# Autodesk Inventor assembly: Eje con costillas
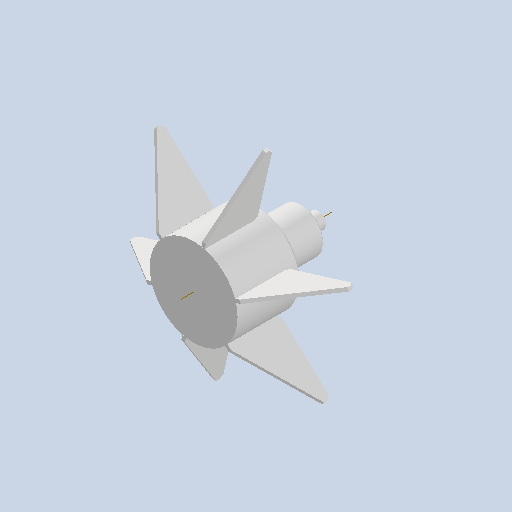
[picture p0: Inventor's stored thumbnail of the model, 512x512]
Saved by Autodesk Inventor 2024.3 (Build 283343000, 343)
## iProperties
Created: 2025-07-04
Part Number: Eje con costillas
Document SubType Name: Assembly
Designer: Daniel Rodriguez
Author: Daniel Rodriguez
## Documents named in this file (3)
- C:\Users\Daniel Rodriguez\Downloads\winch-drum-welding-assembly\Nuestro Winch\Eje con costillas.iam
- C:\Users\Daniel Rodriguez\Downloads\winch-drum-welding-assembly\Nuestro Winch\eje (bolt).ipt
- C:\Users\Daniel Rodriguez\Downloads\winch-drum-welding-assembly\Nuestro Winch\Costilla (rib).ipt
## Components (7 placed, 2 different names)
1. eje (bolt):1 — Nivelación:1, Tangente:1, Coincidencia:1
2. Costilla (rib):1 — Nivelación:1, Tangente:1
3. Costilla (rib):2
4. Costilla (rib):3
5. Costilla (rib):4
6. Costilla (rib):5
7. Costilla (rib):6
## Component patterns: (6 elements, first: Costilla (rib):1)
## Relationships (3: Flush 1, Tangent 1, Mate 1)
- Nivelación:1 [Flush]: eje (bolt):1 ↔ Costilla (rib):1
- Tangente:1: eje (bolt):1 ↔ Costilla (rib):1
- Coincidencia:1 [Mate]: eje (bolt):1
